# Autodesk Inventor assembly: Mirror_on_carriage
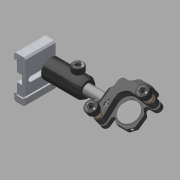
[picture p0: Inventor's stored thumbnail of the model, 180x180]
Saved by Autodesk Inventor 2018 (Build 220112000, 112)
## iProperties
Created: 2018-09-17
Part Number: Mirror_on_carriage
Document SubType Name: Assembly
Designer: Robert Campbell
Author: Robert Campbell
## Documents named in this file (5)
- \\Mac\Home\Dropbox\home\work\Microscopes\SWC_Optics_course_2018\Mirror_on_carriage.iam
- \\Mac\Home\Downloads\LaserAlignment\KM100CP_M-Solidworks.ipt
- \\Mac\Home\Downloads\LaserAlignment\TR50_M-Solidworks.ipt
- \\Mac\Home\Downloads\LaserAlignment\PH50_M-Solidworks.ipt
- \\Mac\Home\Downloads\LaserAlignment\XT66C4-Step.ipt
## Components (4 placed, 4 different names)
1. KM100CP_M-Solidworks:1 — Mate:1, Mate:2
2. TR50_M-Solidworks:1 — Mate:1, Mate:2, Mate:3, Mate:4
3. PH50_M-Solidworks:1 — Mate:3, Mate:4, Mate:5, Mate:6, Angle:1
4. XT66C4-Step:1 — Mate:5, Mate:6, Angle:1
## Relationships (7: Mate 6, Angle 1)
- Mate:1: KM100CP_M-Solidworks:1 ↔ TR50_M-Solidworks:1
- Mate:2: KM100CP_M-Solidworks:1 ↔ TR50_M-Solidworks:1
- Mate:3: TR50_M-Solidworks:1 ↔ PH50_M-Solidworks:1
- Mate:4 (20 mm): TR50_M-Solidworks:1 ↔ PH50_M-Solidworks:1
- Mate:5: PH50_M-Solidworks:1 ↔ XT66C4-Step:1
- Mate:6: PH50_M-Solidworks:1 ↔ XT66C4-Step:1
- Angle:1 (0 deg): PH50_M-Solidworks:1 ↔ XT66C4-Step:1
